# Autodesk Inventor assembly: Propeller and Support Motor Assembly
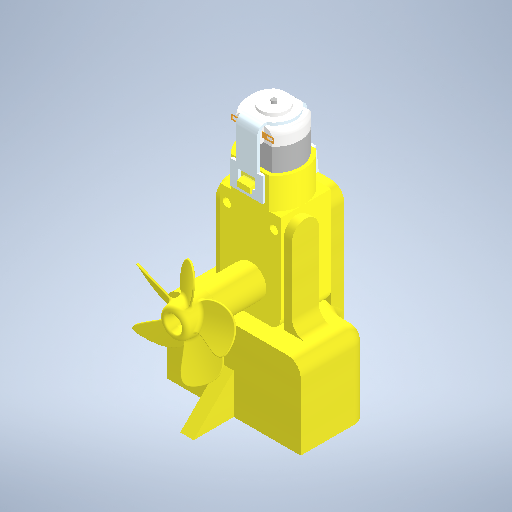
[picture p0: Inventor's stored thumbnail of the model, 512x512]
Saved by Autodesk Inventor 2025.3 (Build 293356000, 356)
## iProperties
Created: 2025-12-07
Part Number: Propeller and Support Motor Assembly
Document SubType Name: Assembly
Designer: maxim
Author: maxim
## Documents named in this file (4)
- C:\Users\maxim\OneDrive\Escritorio\Projects\Self Balancing Robot Project\Propeller and Support Motor Assembly.iam
- C:\Users\maxim\OneDrive\Escritorio\Projects\Self Balancing Robot Project\Soporte Motor.ipt
- C:\Users\maxim\OneDrive\Escritorio\Projects\Self Balancing Robot Project\Propellers.ipt
- C:\Users\maxim\Downloads\TT Motor Dual Shaft\TT Motor Dual Shaft\TT Motor Dual Shaft.ipt
## Components (3 placed, 3 different names)
1. Soporte Motor:1 — Mate:3, Mate:4
2. Propellers:1 — Mate:1, Mate:2
3. TT Motor Dual Shaft:1 — Mate:1, Mate:2, Mate:3, Mate:4
## Relationships (4: Mate 4)
- Mate:1: Propellers:1 ↔ TT Motor Dual Shaft:1
- Mate:2: Propellers:1 ↔ TT Motor Dual Shaft:1
- Mate:3: Soporte Motor:1 ↔ TT Motor Dual Shaft:1
- Mate:4: Soporte Motor:1 ↔ TT Motor Dual Shaft:1
